# Autodesk Inventor assembly: GY-BNO055
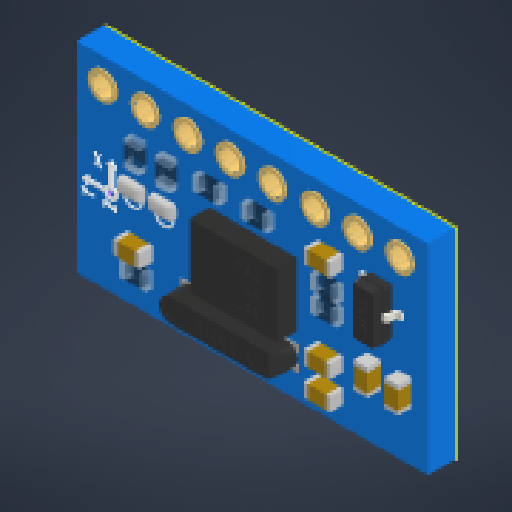
[picture p0: Inventor's stored thumbnail of the model, 512x512]
Saved by Autodesk Inventor 2023 (Build 270158000, 158)
## iProperties
Company: UNSPECIFIED
Created: 1900-01-01
Part Number: GY-BNO055
Description: STEP AP242
Document SubType Name: Assembly
Designer: JV4K
Sending System: C3D Toolkit
Preprocessor: C3D Converter
Title: GY-BNO055
Author: UNSPECIFIED
Revision Number: ANYUNSPECIFIED
## Documents named in this file (8)
- C:\GitHub\Botik\Boards\Aliexpress BNO055\GY-BNO055.iam
- C:\GitHub\Botik\Boards\Aliexpress BNO055\GY-BNO055_PLATE.ipt
- C:\GitHub\Botik\Boards\Aliexpress BNO055\BNO055_CHIP.ipt
- C:\GitHub\Botik\Boards\Aliexpress BNO055\EAML.ipt
- C:\GitHub\Botik\Boards\Aliexpress BNO055\SOLID.ipt
- C:\GitHub\Botik\Boards\Aliexpress BNO055\0603 Resistor.ipt
- C:\GitHub\Botik\Boards\Aliexpress BNO055\0603 Capacitor.ipt
- C:\GitHub\Botik\Boards\Aliexpress BNO055\Перемычка_SMD.ipt
## Components (19 placed, 1 different names)
1. ANY
2. ANY:1 — Заподлицо:1, Заподлицо:2
3. ANY:2
4. ANY:3
5. ANY:4
6. ANY:5
7. ANY:6
8. ANY:7
9. ANY:8
10. ANY:9
11. ANY:10
12. ANY:11
13. ANY:12
14. ANY:13
15. ANY:14
16. ANY:15
17. ANY:16
18. ANY:17
19. ANY:18
## Relationships (4: Flush 2, Mate 2)
- Заподлицо:1 [Flush] (-1.9 mm): ANY:1
- Заподлицо:2 [Flush] (-2.6 mm): ANY:1
- Совмещение:1 [Mate]
- Совмещение:2 [Mate]
